# Autodesk Inventor assembly: 42025144
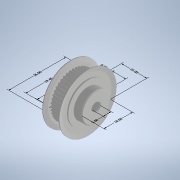
[picture p0: Inventor's stored thumbnail of the model, 180x180]
Saved by Autodesk Inventor 2021 (Build 250183000, 183)
## iProperties
Category: PARTsolutions
Company: CHIARAVALLI
Created: 2025-04-22
Part Number: 42025144
Catalog Web Link: www.cadenas.de
Description: MXL 025-Timing pulleys with pilot bore
Vendor: CHIARAVALLI
Document SubType Name: Assembly
Designer: psAdmin
Manufacturer: CHIARAVALLI
Mass: 30 g
Surface Area: 52.1841 cm^2
Volume: 7.62027 cm^3
Density: 3.93687 g/cm^3
Title: 42025144
Author: Cadenas PARTsolutions
Comments: Timing pulleys with pilot bore
PSOL_IDENT_0: {$CADENAS_DATA/23d-libs/chiaravalli/open_transmission/toothed_pulleys/timing_pulleys_with_pilot_bore
PSOL_IDENT_1: /mxl/mxl_025_aluminium_asmtab.prj},172 {VTYP=3D},{STYP=ASSTAB},{NB=42025144},{LINA=42025144},{NN=MXL
PSOL_IDENT_2: 025},{DATE=05.08.2024 16:01:07},{GEOMDATE=18.04.2024 11:10:43},{VERSION=},{LINEID=120},{WBVAR=},{WB
PSOL_IDENT_3: NUMERIC=}  {NB=42025144},{LINA=42025144},{KT=DUMMY},{TYPE=44 MXL 025},{CODE=42025144},{T=44},{EXEC=1
PSOL_IDENT_4: F},{DP=28.46},{DE=27.95},{DF=36},{DM=18},{DM1=-},{F=11.0},{L=16},{D=5},{NF=510},{WEIGHT=0.03},{MAT=A
PSOL_IDENT_5: LUMINIUM},{DX=5},{NFX=510},{DM1X=0.0},{L1=25.0},{PPATH=mxl_025_aluminium_asmtpl.prj}
NB: 42025144
NN: MXL 025
NT: Timing pulleys with pilot bore
NBSYN: $CODE.
LINA: 42025144
CATALOG: Chiaravalli
TYPE: 44 MXL 025
CODE: 42025144
T: 44
EXEC: 1F
DP: 28.46
DE: 27.95
DF: 36
DM: 18
F: 11
L: 16
D: 5
NF: 510
WEIGHT: 0.03
MAT: Aluminum
SUPPLIER: CHIARAVALLI
ARTICLENO: 42025144
BOMINFO: 42025144
CREATOR: CADENAS GmbH
## Documents named in this file (3)
- e:\temp\worker_COMMON_160\temp\tmp_960_108_ldTkQ\format_0\42025144.iam
- e:\temp\worker_COMMON_160\temp\tmp_960_108_ldTkQ\format_0\4202514444.ipt
- e:\temp\worker_COMMON_160\temp\tmp_960_108_ldTkQ\format_0\49200510.ipt
## Components (3 placed, 2 different names)
1. 4202514444:1 — FLL_XY@1 <-> FL1_XY@2, FLL_Z@1 <-> FL1_Z@2, FLL_YZ@1 <-> FL1_YZ@2, FLR_XY@1 <-> FL1_XY@3, FLR_Z@1 <-> FL1_Z@3, FLR_YZ@1 <-> FL1_YZ@3
2. 49200510:1 — FLL_XY@1 <-> FL1_XY@2, FLL_Z@1 <-> FL1_Z@2, FLL_YZ@1 <-> FL1_YZ@2
3. 49200510:2 — FLR_XY@1 <-> FL1_XY@3, FLR_Z@1 <-> FL1_Z@3, FLR_YZ@1 <-> FL1_YZ@3
## Relationships (6: Mate 4, Angle 2)
- FLL_XY@1 <-> FL1_XY@2 [Mate]: 4202514444:1 ↔ 49200510:1
- FLL_Z@1 <-> FL1_Z@2 [Mate]: 4202514444:1 ↔ 49200510:1
- FLL_YZ@1 <-> FL1_YZ@2 [Angle] (90 deg): 4202514444:1 ↔ 49200510:1
- FLR_XY@1 <-> FL1_XY@3 [Mate]: 4202514444:1 ↔ 49200510:2
- FLR_Z@1 <-> FL1_Z@3 [Mate]: 4202514444:1 ↔ 49200510:2
- FLR_YZ@1 <-> FL1_YZ@3 [Angle] (90 deg): 4202514444:1 ↔ 49200510:2
